# Autodesk Inventor assembly: MG-Dribbler Seite v2
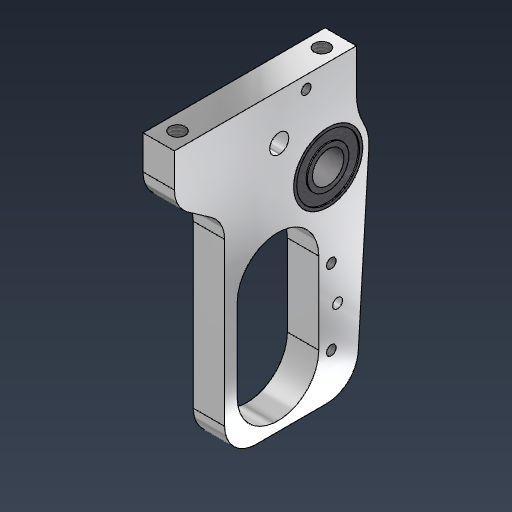
[picture p0: Inventor's stored thumbnail of the model, 512x512]
Saved by Autodesk Inventor 2022.3 (Build 263350000, 350)
## iProperties
Part Number: MG-Dribbler Seite v2
Material: Generisch
Document SubType Name: Assembly
Designer: rYan
Mass: 12.7765 g
Surface Area: 33.8166 cm^2
Volume: 4.0468 cm^3
Author: rYan
## Documents named in this file (3)
- D:\TIGERsGIT\Hardware\mechanik\2020\Inventor\Robot\Dribbler\MG-Dribbler Seite v2.iam
- D:\TIGERsGIT\Hardware\mechanik\2020\Inventor\Purchased Parts\Kugellager 685-ZZ-C3.ipt
- D:\TIGERsGIT\Hardware\mechanik\2020\Inventor\Robot\Dribbler\Dribbler Seite v2.ipt
## Components (2 placed, 2 different names)
1. Dribbler Seite v2:1 — Einfügen:1
2. Kugellager 685-ZZ-C3:1 — Einfügen:1
## Relationships (1: Insert 1)
- Einfügen:1 [Insert]: Dribbler Seite v2:1 ↔ Kugellager 685-ZZ-C3:1
